# Autodesk Inventor assembly: Assembly4
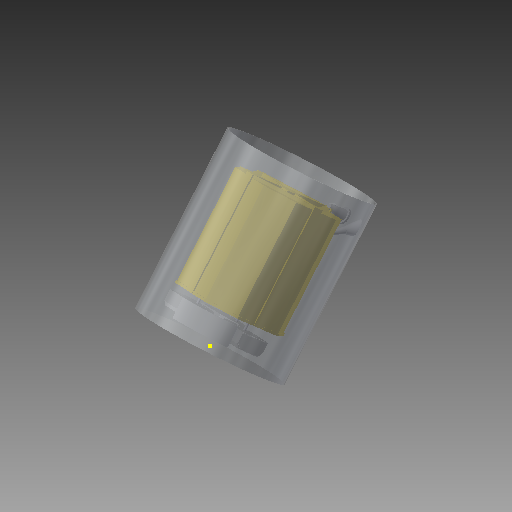
[picture p0: Inventor's stored thumbnail of the model, 512x512]
Saved by Autodesk Inventor 2018 (Build 220112000, 112)
## iProperties
Created: 2021-03-17
Part Number: Assembly4
Document SubType Name: Assembly
Designer: dell
Author: dell
## Documents named in this file (4)
- D:\Autodesk\Projects\C-C\a1\ES101 GROUP-13 PROJECT\FINAL MODEL\Resolved files\Assembly4.iam
- D:\Autodesk\Projects\C-C\a1\ES101 GROUP-13 PROJECT\INDIVIDUAL WORK\Tejas\Resolved files\Derived Gyros.ipt
- D:\Autodesk\Projects\C-C\a1\ES101 GROUP-13 PROJECT\FINAL MODEL\Resolved files\Assembly3.iam
- D:\Autodesk\Projects\C-C\a1\ES101 GROUP-13 PROJECT\INDIVIDUAL WORK\Tejas\Resolved files\Derived Gyros_MIR.ipt
## Components (3 placed, 3 different names)
1. Derived Gyros:1 — Tangent:1
2. Assembly3:1 [sub-assembly] — Tangent:1
3. Derived Gyros_MIR:1
## Relationships (1: Tangent 1)
- Tangent:1: Derived Gyros:1 ↔ Assembly3:1
